# Autodesk Inventor assembly: tinyboy
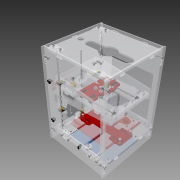
[picture p0: Inventor's stored thumbnail of the model, 180x180]
Saved by Autodesk Inventor 2013 (Build 170138000, 138)
## iProperties
Created: 2015-02-19
Part Number: tinyboy
Document SubType Name: Assembly
Designer: Noa Izumi
Author: Noa Izumi
## Documents named in this file (20)
- C:\reprap\TinyBoy_v3_20150222\tinyboy.iam
- C:\reprap\TinyBoy_v3_20150222\assembly base.iam
- C:\reprap\TinyBoy_v3_20150222\plastic_part_01.ipt
- C:\reprap\TinyBoy_v3_20150222\plastic_part_02.ipt
- C:\reprap\TinyBoy_v3_20150222\plastic_part_03.ipt
- C:\reprap\TinyBoy_v3_20150222\plastic_part_05.ipt
- C:\reprap\TinyBoy_v3_20150222\plastic_part_00.ipt
- C:\reprap\TinyBoy_v3_20150222\screw_M3_6_hex.ipt
- C:\reprap\TinyBoy_v3_20150222\rod_M4_140.ipt
- C:\reprap\TinyBoy_v3_20150222\screw_M3_12_hex.ipt
- C:\reprap\TinyBoy_v3_20150222\rod_M4_180.ipt
- C:\reprap\TinyBoy_v3_20150222\nut_M3.ipt
- C:\reprap\TinyBoy_v3_20150222\assembly y.iam
- C:\reprap\TinyBoy_v3_20150222\assembly z.iam
- C:\reprap\TinyBoy_v3_20150222\assembly extruder.iam
- C:\reprap\TinyBoy_v3_20150222\z_shaft.iam
- C:\reprap\TinyBoy_v3_20150222\assembly x.iam
- C:\reprap\TinyBoy_v3_20150222\screw_M4_8_hex.ipt
- C:\reprap\TinyBoy_v3_20150222\fastener_03.ipt
- C:\reprap\TinyBoy_v3_20150222\fastener_04.ipt
## Components (59 placed, 19 different names)
1. assembly base:1 [sub-assembly] — 齊平:1, 齊平:2, 貼合:1, 齊平:3, 貼合:2, 齊平:4, 插入:35, 插入:36, 角度:9, 插入:47
2. plastic_part_02:1 — 齊平:8, 貼合:4, 齊平:11, 插入:27, 插入:28, 插入:29, 插入:30, 齊平:12
3. plastic_part_03:1 — 插入:9, 插入:10, 插入:11, 插入:12, 齊平:1, 齊平:2, 貼合:1, 齊平:5, 貼合:3, 齊平:8, 貼合:4, 齊平:9, 齊平:10, 貼合:5, 插入:25, 插入:26, 齊平:11, 角度:1, 角度:2, 角度:3, 角度:4, 角度:10, 角度:11, 角度:12, 貼合:6, 貼合:7, 貼合:8, 貼合:12, 貼合:13, 貼合:14, 貼合:15, 貼合:16, 貼合:17
4. plastic_part_03:2 — 插入:17, 插入:18, 插入:19, 插入:20, 齊平:3, 貼合:2, 齊平:4, 角度:5, 角度:6, 角度:7, 角度:8, 貼合:9, 貼合:10, 貼合:11, 貼合:18, 貼合:19, 貼合:20, 貼合:21, 貼合:22, 貼合:23
5. plastic_part_05:1 — 插入:1, 插入:2, 插入:3, 插入:4, 齊平:5, 貼合:3, 齊平:12
6. plastic_part_00:1 — 插入:9, 插入:10, 插入:13, 插入:14
7. plastic_part_00:2 — 插入:1, 插入:2, 插入:5, 插入:6
8. plastic_part_00:3 — 插入:11, 插入:12, 插入:15, 插入:16
9. plastic_part_00:4 — 插入:3, 插入:4, 插入:7, 插入:8
10. plastic_part_00:5 — 插入:17, 插入:18, 插入:23, 插入:24
11. plastic_part_00:6 — 插入:19, 插入:20, 插入:21, 插入:22
12. screw_M3_6_hex:1 — 插入:8
13. screw_M3_6_hex:2 — 插入:6
14. screw_M3_6_hex:3 — 插入:7
15. screw_M3_6_hex:4 — 插入:5
16. screw_M3_6_hex:5 — 插入:21
17. screw_M3_6_hex:6 — 插入:22
18. screw_M3_6_hex:7 — 插入:13
19. screw_M3_6_hex:8 — 插入:14
20. screw_M3_6_hex:9 — 插入:15
21. screw_M3_6_hex:10 — 插入:16
22. screw_M3_6_hex:11 — 插入:23
23. screw_M3_6_hex:12 — 插入:24
24. plastic_part_01:1 — 齊平:9, 齊平:10, 貼合:5, 插入:31, 插入:32, 插入:33, 插入:34, 插入:45, 插入:46
25. rod_M4_140:1 — 插入:25, 相切:1
26. rod_M4_140:2 — 插入:26
27. screw_M3_12_hex:1 — 插入:29, 插入:44
28. screw_M3_12_hex:2 — 插入:31, 插入:37
29. screw_M3_12_hex:3 — 插入:32, 插入:42
30. screw_M3_12_hex:4 — 插入:27, 插入:39
31. screw_M3_12_hex:5 — 插入:28, 插入:40
32. screw_M3_12_hex:6 — 插入:33, 插入:38
33. screw_M3_12_hex:7 — 插入:30, 插入:41
34. screw_M3_12_hex:8 — 插入:34, 插入:43
35. rod_M4_180:1 — 插入:36
36. rod_M4_180:2 — 插入:35, 相切:2
37. nut_M3:1 — 插入:37, 角度:2
38. nut_M3:2 — 插入:44, 角度:7
39. nut_M3:3 — 插入:38, 角度:4
40. nut_M3:4 — 插入:43, 角度:8
41. nut_M3:5 — 插入:42, 角度:5
42. nut_M3:6 — 插入:40, 角度:3
43. nut_M3:7 — 插入:41, 角度:6
44. nut_M3:8 — 插入:39, 角度:1
45. assembly y:1 [sub-assembly] — 角度:9, 相切:1, 角度:10
46. assembly z:1 [sub-assembly] — 相切:2, 角度:11, 角度:12, 相切:3, 角度:13, 角度:14
47. assembly extruder:1 [sub-assembly] — 插入:45, 插入:46, 插入:48, 插入:49, 插入:50, 插入:51
48. z_shaft:1 [sub-assembly] — 插入:47
49. assembly x:1 [sub-assembly] — 相切:3, 角度:13, 角度:14
50. screw_M4_8_hex:1 — 插入:48
51. screw_M4_8_hex:2 — 插入:51
52. screw_M4_8_hex:3 — 插入:50
53. screw_M4_8_hex:4 — 插入:49
54. fastener_03:1 — 貼合:6, 貼合:7, 貼合:8
55. fastener_03:2 — 貼合:9, 貼合:10, 貼合:11
56. fastener_04:1 — 貼合:12, 貼合:13, 貼合:14
57. fastener_04:2 — 貼合:15, 貼合:16, 貼合:17
58. fastener_04:3 — 貼合:19, 貼合:21, 貼合:23
59. fastener_04:4 — 貼合:18, 貼合:20, 貼合:22
## Relationships (101: Insert 51, Mate 23, Angle 14, Flush 10, Tangent 3)
- 插入:1 [Insert]: plastic_part_05:1 ↔ plastic_part_00:2
- 插入:2 [Insert]: plastic_part_05:1 ↔ plastic_part_00:2
- 插入:3 [Insert]: plastic_part_05:1 ↔ plastic_part_00:4
- 插入:4 [Insert]: plastic_part_05:1 ↔ plastic_part_00:4
- 插入:5 [Insert]: plastic_part_00:2 ↔ screw_M3_6_hex:4
- 插入:6 [Insert]: plastic_part_00:2 ↔ screw_M3_6_hex:2
- 插入:7 [Insert]: plastic_part_00:4 ↔ screw_M3_6_hex:3
- 插入:8 [Insert]: plastic_part_00:4 ↔ screw_M3_6_hex:1
- 插入:9 [Insert]: plastic_part_03:1 ↔ plastic_part_00:1
- 插入:10 [Insert]: plastic_part_03:1 ↔ plastic_part_00:1
- 插入:11 [Insert]: plastic_part_03:1 ↔ plastic_part_00:3
- 插入:12 [Insert]: plastic_part_03:1 ↔ plastic_part_00:3
- 插入:13 [Insert]: plastic_part_00:1 ↔ screw_M3_6_hex:7
- 插入:14 [Insert]: plastic_part_00:1 ↔ screw_M3_6_hex:8
- 插入:15 [Insert]: plastic_part_00:3 ↔ screw_M3_6_hex:9
- 插入:16 [Insert]: plastic_part_00:3 ↔ screw_M3_6_hex:10
- 插入:17 [Insert]: plastic_part_03:2 ↔ plastic_part_00:5
- 插入:18 [Insert]: plastic_part_03:2 ↔ plastic_part_00:5
- 插入:19 [Insert]: plastic_part_03:2 ↔ plastic_part_00:6
- 插入:20 [Insert]: plastic_part_03:2 ↔ plastic_part_00:6
- 插入:21 [Insert]: plastic_part_00:6 ↔ screw_M3_6_hex:5
- 插入:22 [Insert]: plastic_part_00:6 ↔ screw_M3_6_hex:6
- 插入:23 [Insert]: plastic_part_00:5 ↔ screw_M3_6_hex:11
- 插入:24 [Insert]: plastic_part_00:5 ↔ screw_M3_6_hex:12
- 齊平:1 [Flush]: assembly base:1 ↔ plastic_part_03:1
- 齊平:2 [Flush]: assembly base:1 ↔ plastic_part_03:1
- 貼合:1 [Mate]: assembly base:1 ↔ plastic_part_03:1
- 齊平:3 [Flush]: assembly base:1 ↔ plastic_part_03:2
- 貼合:2 [Mate]: assembly base:1 ↔ plastic_part_03:2
- 齊平:4 [Flush]: assembly base:1 ↔ plastic_part_03:2
- 齊平:5 [Flush]: plastic_part_03:1 ↔ plastic_part_05:1
- 貼合:3 [Mate]: plastic_part_03:1 ↔ plastic_part_05:1
- 齊平:8 [Flush]: plastic_part_02:1 ↔ plastic_part_03:1
- 貼合:4 [Mate]: plastic_part_02:1 ↔ plastic_part_03:1
- 齊平:9 [Flush]: plastic_part_03:1 ↔ plastic_part_01:1
- 齊平:10 [Flush]: plastic_part_03:1 ↔ plastic_part_01:1
- 貼合:5 [Mate]: plastic_part_03:1 ↔ plastic_part_01:1
- 插入:25 [Insert]: plastic_part_03:1 ↔ rod_M4_140:1
- 插入:26 [Insert]: plastic_part_03:1 ↔ rod_M4_140:2
- 齊平:11 [Flush]: plastic_part_02:1 ↔ plastic_part_03:1
- 插入:27 [Insert]: plastic_part_02:1 ↔ screw_M3_12_hex:4
- 插入:28 [Insert]: plastic_part_02:1 ↔ screw_M3_12_hex:5
- 插入:29 [Insert]: plastic_part_02:1 ↔ screw_M3_12_hex:1
- 插入:30 [Insert]: plastic_part_02:1 ↔ screw_M3_12_hex:7
- 插入:31 [Insert]: plastic_part_01:1 ↔ screw_M3_12_hex:2
- 插入:32 [Insert]: plastic_part_01:1 ↔ screw_M3_12_hex:3
- 插入:33 [Insert]: plastic_part_01:1 ↔ screw_M3_12_hex:6
- 插入:34 [Insert]: plastic_part_01:1 ↔ screw_M3_12_hex:8
- 插入:35 [Insert]: assembly base:1 ↔ rod_M4_180:2
- 插入:36 [Insert]: assembly base:1 ↔ rod_M4_180:1
- 插入:37 [Insert]: screw_M3_12_hex:2 ↔ nut_M3:1
- 插入:38 [Insert]: screw_M3_12_hex:6 ↔ nut_M3:3
- 插入:39 [Insert]: screw_M3_12_hex:4 ↔ nut_M3:8
- 插入:40 [Insert]: screw_M3_12_hex:5 ↔ nut_M3:6
- 插入:41 [Insert]: screw_M3_12_hex:7 ↔ nut_M3:7
- 插入:42 [Insert]: screw_M3_12_hex:3 ↔ nut_M3:5
- 插入:43 [Insert]: screw_M3_12_hex:8 ↔ nut_M3:4
- 插入:44 [Insert]: screw_M3_12_hex:1 ↔ nut_M3:2
- 角度:1 [Angle] (0 deg): plastic_part_03:1 ↔ nut_M3:8
- 角度:2 [Angle] (0 deg): plastic_part_03:1 ↔ nut_M3:1
- 角度:3 [Angle] (0 deg): plastic_part_03:1 ↔ nut_M3:6
- 角度:4 [Angle] (0 deg): plastic_part_03:1 ↔ nut_M3:3
- 角度:5 [Angle] (0 deg): plastic_part_03:2 ↔ nut_M3:5
- 角度:6 [Angle] (0 deg): plastic_part_03:2 ↔ nut_M3:7
- 角度:7 [Angle] (0 deg): plastic_part_03:2 ↔ nut_M3:2
- 角度:8 [Angle] (0 deg): plastic_part_03:2 ↔ nut_M3:4
- 角度:9 [Angle] (0 deg): assembly base:1 ↔ assembly y:1
- 相切:1 [Tangent]: rod_M4_140:1 ↔ assembly y:1
- 角度:10 [Angle] (0 deg): plastic_part_03:1 ↔ assembly y:1
- 相切:2 [Tangent]: rod_M4_180:2 ↔ assembly z:1
- 角度:11 [Angle] (0 deg): plastic_part_03:1 ↔ assembly z:1
- 角度:12 [Angle] (0 deg): plastic_part_03:1 ↔ assembly z:1
- 插入:45 [Insert]: plastic_part_01:1 ↔ assembly extruder:1
- 插入:46 [Insert]: plastic_part_01:1 ↔ assembly extruder:1
- 插入:47 [Insert]: assembly base:1 ↔ z_shaft:1
- 相切:3 [Tangent]: assembly z:1 ↔ assembly x:1
- 角度:13 [Angle] (0 deg): assembly z:1 ↔ assembly x:1
- 角度:14 [Angle] (0 deg): assembly z:1 ↔ assembly x:1
- 插入:48 [Insert]: assembly extruder:1 ↔ screw_M4_8_hex:1
- 插入:49 [Insert]: assembly extruder:1 ↔ screw_M4_8_hex:4
- 插入:50 [Insert]: assembly extruder:1 ↔ screw_M4_8_hex:3
- 插入:51 [Insert]: assembly extruder:1 ↔ screw_M4_8_hex:2
- 貼合:6 [Mate]: plastic_part_03:1 ↔ fastener_03:1
- 貼合:7 [Mate]: plastic_part_03:1 ↔ fastener_03:1
- 貼合:8 [Mate]: plastic_part_03:1 ↔ fastener_03:1
- 貼合:9 [Mate]: plastic_part_03:2 ↔ fastener_03:2
- 貼合:10 [Mate]: plastic_part_03:2 ↔ fastener_03:2
- 貼合:11 [Mate]: plastic_part_03:2 ↔ fastener_03:2
- 貼合:12 [Mate]: plastic_part_03:1 ↔ fastener_04:1
- 貼合:13 [Mate]: plastic_part_03:1 ↔ fastener_04:1
- 貼合:14 [Mate]: plastic_part_03:1 ↔ fastener_04:1
- 貼合:15 [Mate]: plastic_part_03:1 ↔ fastener_04:2
- 貼合:16 [Mate]: plastic_part_03:1 ↔ fastener_04:2
- 貼合:17 [Mate]: plastic_part_03:1 ↔ fastener_04:2
- 貼合:18 [Mate]: plastic_part_03:2 ↔ fastener_04:4
- 貼合:19 [Mate]: plastic_part_03:2 ↔ fastener_04:3
- 貼合:20 [Mate]: plastic_part_03:2 ↔ fastener_04:4
- 貼合:21 [Mate]: plastic_part_03:2 ↔ fastener_04:3
- 貼合:22 [Mate]: plastic_part_03:2 ↔ fastener_04:4
- 貼合:23 [Mate]: plastic_part_03:2 ↔ fastener_04:3
- 齊平:12 [Flush]: plastic_part_02:1 ↔ plastic_part_05:1
